# Autodesk Inventor assembly: Disk F Assembly
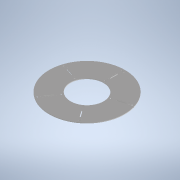
[picture p0: Inventor's stored thumbnail of the model, 180x180]
Saved by Autodesk Inventor 2020 (Build 240168000, 168)
## iProperties
Created: 2020-05-11
Part Number: Disk F Assembly
Document SubType Name: Assembly
Designer: Dan Wikman
Author: Dan Wikman
## Documents named in this file (6)
- C:\Users\Dan Wikman\OneDrive\University Life\2020, Semester 1\METR4900 Honours Thesis\Full Scale Design\Disk F Assembly.iam
- C:\Users\Dan Wikman\OneDrive\University Life\2020, Semester 1\METR4900 Honours Thesis\Full Scale Design\Platform F1.ipt
- C:\Users\Dan Wikman\OneDrive\University Life\2020, Semester 1\METR4900 Honours Thesis\Full Scale Design\Platform F2.ipt
- C:\Users\Dan Wikman\OneDrive\University Life\2020, Semester 1\METR4900 Honours Thesis\Full Scale Design\Platform F3.ipt
- C:\Users\Dan Wikman\OneDrive\University Life\2020, Semester 1\METR4900 Honours Thesis\Full Scale Design\Platform F4.ipt
- C:\Users\Dan Wikman\OneDrive\University Life\2020, Semester 1\METR4900 Honours Thesis\Full Scale Design\Platform F5.ipt
## Components (5 placed, 5 different names)
1. Platform F1:1 — Flush:1, Mate:1, Mate:2, Mate:3, Mate:4
2. Platform F2:1 — Flush:1, Flush:2, Mate:1, Mate:2, Mate:7
3. Platform F3:1 — Flush:2, Flush:3, Mate:3, Mate:4, Mate:5, Mate:6
4. Platform F4:1 — Flush:3, Flush:4, Mate:5, Mate:6, Mate:8
5. Platform F5:1 — Flush:4, Mate:7, Mate:8
## Relationships (12: Mate 8, Flush 4)
- Flush:1: Platform F1:1 ↔ Platform F2:1
- Flush:2: Platform F2:1 ↔ Platform F3:1
- Flush:3: Platform F3:1 ↔ Platform F4:1
- Flush:4: Platform F4:1 ↔ Platform F5:1
- Mate:1: Platform F1:1 ↔ Platform F2:1
- Mate:2: Platform F1:1 ↔ Platform F2:1
- Mate:3: Platform F1:1 ↔ Platform F3:1
- Mate:4: Platform F1:1 ↔ Platform F3:1
- Mate:5: Platform F3:1 ↔ Platform F4:1
- Mate:6: Platform F3:1 ↔ Platform F4:1
- Mate:7: Platform F2:1 ↔ Platform F5:1
- Mate:8: Platform F4:1 ↔ Platform F5:1
